# Autodesk Inventor assembly: PcbBoard_last3
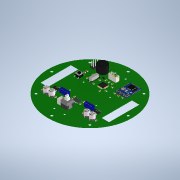
[picture p0: Inventor's stored thumbnail of the model, 180x180]
Saved by Autodesk Inventor 2020 (Build 240168000, 168)
## iProperties
Company: Open CASCADE
Created: 2020-05-07
Part Number: PcbBoard_last3
Description: Open CASCADE Model
Document SubType Name: Assembly
Designer: jamnissa
Authority: Unknown
Mass: 7.39378 g
Surface Area: 248.728 cm^2
Volume: 7.39378 cm^3
Density: 1 g/cm^3
Sending System: Open CASCADE 6.8
Preprocessor: Open CASCADE STEP processor 6.8
Title: Open CASCADE Shape Model
Author: Author
## Documents named in this file (45)
- C:\Users\jama1\Documents\GitHub\JRobots\pcbCase\Board\PcbBoard_last3.iam
- C:\Users\jama1\Documents\GitHub\JRobots\pcbCase\Board\Board.iam
- C:\Users\jama1\Documents\GitHub\JRobots\pcbCase\Board\DD2.iam
- C:\Users\jama1\Documents\GitHub\JRobots\pcbCase\Board\C15.iam
- C:\Users\jama1\Documents\GitHub\JRobots\pcbCase\Board\BQ1.iam
- C:\Users\jama1\Documents\GitHub\JRobots\pcbCase\Board\XS4.iam
- C:\Users\jama1\Documents\GitHub\JRobots\pcbCase\Board\XS3.iam
- C:\Users\jama1\Documents\GitHub\JRobots\pcbCase\Board\XS2.iam
- C:\Users\jama1\Documents\GitHub\JRobots\pcbCase\Board\XP1.iam
- C:\Users\jama1\Documents\GitHub\JRobots\pcbCase\Board\XS1.iam
- C:\Users\jama1\Documents\GitHub\JRobots\pcbCase\Board\VT1.iam
- C:\Users\jama1\Documents\GitHub\JRobots\pcbCase\Board\VD1.iam
- C:\Users\jama1\Documents\GitHub\JRobots\pcbCase\Board\SW2.iam
- C:\Users\jama1\Documents\GitHub\JRobots\pcbCase\Board\SW1.iam
- C:\Users\jama1\Documents\GitHub\JRobots\pcbCase\Board\R6.iam
- C:\Users\jama1\Documents\GitHub\JRobots\pcbCase\Board\R5.iam
- C:\Users\jama1\Documents\GitHub\JRobots\pcbCase\Board\R4.iam
- C:\Users\jama1\Documents\GitHub\JRobots\pcbCase\Board\R3.iam
- C:\Users\jama1\Documents\GitHub\JRobots\pcbCase\Board\R2.iam
- C:\Users\jama1\Documents\GitHub\JRobots\pcbCase\Board\R1.iam
- C:\Users\jama1\Documents\GitHub\JRobots\pcbCase\Board\L1.iam
- C:\Users\jama1\Documents\GitHub\JRobots\pcbCase\Board\DD3.iam
- C:\Users\jama1\Documents\GitHub\JRobots\pcbCase\Board\DD1.iam
- C:\Users\jama1\Documents\GitHub\JRobots\pcbCase\Board\DA2.iam
- C:\Users\jama1\Documents\GitHub\JRobots\pcbCase\Board\DA1.iam
- C:\Users\jama1\Documents\GitHub\JRobots\pcbCase\Board\C19.iam
- C:\Users\jama1\Documents\GitHub\JRobots\pcbCase\Board\C18.iam
- C:\Users\jama1\Documents\GitHub\JRobots\pcbCase\Board\C17.iam
- C:\Users\jama1\Documents\GitHub\JRobots\pcbCase\Board\C16.iam
- C:\Users\jama1\Documents\GitHub\JRobots\pcbCase\Board\C14.iam
- C:\Users\jama1\Documents\GitHub\JRobots\pcbCase\Board\C13.iam
- C:\Users\jama1\Documents\GitHub\JRobots\pcbCase\Board\C12.iam
- C:\Users\jama1\Documents\GitHub\JRobots\pcbCase\Board\C11.iam
- C:\Users\jama1\Documents\GitHub\JRobots\pcbCase\Board\C10.iam
- C:\Users\jama1\Documents\GitHub\JRobots\pcbCase\Board\C9.iam
- C:\Users\jama1\Documents\GitHub\JRobots\pcbCase\Board\C8.iam
- C:\Users\jama1\Documents\GitHub\JRobots\pcbCase\Board\C7.iam
- C:\Users\jama1\Documents\GitHub\JRobots\pcbCase\Board\C6.iam
- C:\Users\jama1\Documents\GitHub\JRobots\pcbCase\Board\C5.iam
- C:\Users\jama1\Documents\GitHub\JRobots\pcbCase\Board\C4.iam
- C:\Users\jama1\Documents\GitHub\JRobots\pcbCase\Board\C3.iam
- C:\Users\jama1\Documents\GitHub\JRobots\pcbCase\Board\C2.iam
- C:\Users\jama1\Documents\GitHub\JRobots\pcbCase\Board\C1.iam
- C:\Users\jama1\Documents\GitHub\JRobots\pcbCase\Board\BQ2.iam
- C:\Users\jama1\Documents\GitHub\JRobots\pcbCase\Board\XP.iam
## Components (45 placed, 45 different names)
1. Board_2 [sub-assembly] — Совмещение:1
2. DD2_6 [sub-assembly]
3. C15_8 [sub-assembly]
4. BQ1_10 [sub-assembly]
5. XS4_12 [sub-assembly]
6. XS3_14 [sub-assembly]
7. XS2_16 [sub-assembly]
8. XP1_18 [sub-assembly]
9. XS1_20 [sub-assembly]
10. VT1_22 [sub-assembly]
11. VD1_24 [sub-assembly]
12. SW2_37 [sub-assembly]
13. SW1_39 [sub-assembly]
14. R6_42 [sub-assembly]
15. R5_45 [sub-assembly]
16. R4_48 [sub-assembly]
17. R3_51 [sub-assembly]
18. R2_54 [sub-assembly]
19. R1_57 [sub-assembly]
20. L1_59 [sub-assembly]
21. DD3_73 [sub-assembly]
22. DD1_75 [sub-assembly]
23. DA2_82 [sub-assembly]
24. DA1_84 [sub-assembly]
25. C19_86 [sub-assembly]
26. C18_88 [sub-assembly]
27. C17_90 [sub-assembly]
28. C16_92 [sub-assembly]
29. C14_94 [sub-assembly]
30. C13_96 [sub-assembly]
31. C12_98 [sub-assembly]
32. C11_100 [sub-assembly]
33. C10_102 [sub-assembly]
34. C9_104 [sub-assembly]
35. C8_106 [sub-assembly]
36. C7_108 [sub-assembly]
37. C6_110 [sub-assembly]
38. C5_112 [sub-assembly]
39. C4_114 [sub-assembly]
40. C3_116 [sub-assembly]
41. C2_118 [sub-assembly]
42. C1_120 [sub-assembly]
43. BQ2_136 [sub-assembly]
44. XP1:2 [sub-assembly]
45. XP:2 [sub-assembly] — Совмещение:1
## Relationships (1: Mate 1)
- Совмещение:1 [Mate]: Board_2 ↔ XP:2
